# Autodesk Inventor assembly: Aufbau1,0
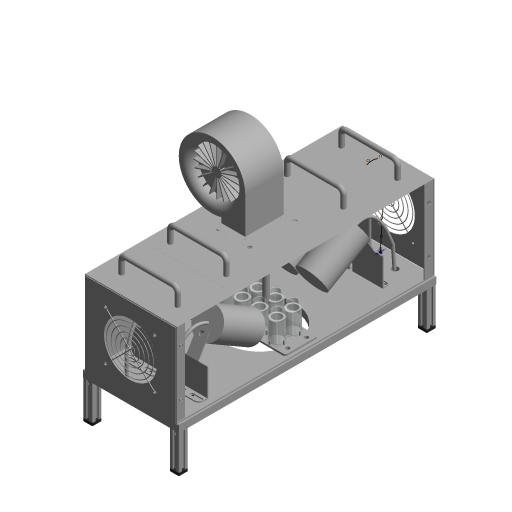
[picture p0: Inventor's stored thumbnail of the model, 512x512]
Saved by Autodesk Inventor 2024 (Build 280153000, 153)
## iProperties
Created: 2021-10-11
Part Number: Aufbau1,0
Document SubType Name: Baugruppe
Designer: bhelg
Author: bhelg
## Documents named in this file (20)
- E:\UV Reaktor 2\Aufbau 2,0.iam
- E:\UV Reaktor 2\Lampe.ipt
- E:\UV Reaktor 2\Glas klein.ipt
- E:\UV Reaktor 2\Grundplatte 2,0.ipt
- E:\UV Reaktor 2\Lampenhalterung 2,0.ipt
- E:\UV Reaktor 2\Halterung Gläser D27.4.ipt
- E:\UV Reaktor 2\Wobatech Abdeckkappe 20x20.ipt
- E:\UV Reaktor 2\20x20Profil 1.0.ipt
- E:\UV Reaktor 2\Deckel1,0.ipt
- E:\UV Reaktor 2\Seitenplatte 1,0.ipt
- E:\UV Reaktor 2\Sensormechanismus\Stativstange.ipt
- E:\UV Reaktor 2\Sensormechanismus\Stellring.ipt
- E:\UV Reaktor 2\Sensormechanismus\Arm.ipt
- E:\UV Reaktor 2\Sensormechanismus\Glashalter.ipt
- E:\UV Reaktor 2\Sensormechanismus\Glas.ipt
- E:\UV Reaktor 2\Blechgriff.ipt
- E:\UV Reaktor 2\Deckelanschlag.ipt
- E:\UV Reaktor 2\Deckel 2,0.ipt
- E:\UV Reaktor 2\Lüfter G1G108-AB17-02 1,0.ipt
- E:\UV Reaktor 2\Lüftergitter 1,0.ipt
## Components (45 placed, 19 different names)
1. Grundplatte 2,0:1 — Fluchtend:1, Fluchtend:2, Fluchtend:3, Passend:1, Winkel:1, Passend:3, Winkel:2, Einfügen:3, Tangential:1, Passend:8, Passend:9, Passend:10, Winkel:3, Winkel:4, Winkel:5, Tangential:2, Tangential:3, Tangential:4, Passend:22, Passend:23, Passend:24, Passend:25, Einfügen:19, Einfügen:20, Einfügen:21, Einfügen:22, Winkel:6, Passend:31, Passend:32, Winkel:7, Winkel:8, Einfügen:25, Fluchtend:5, Fluchtend:6
2. Lampenhalterung 2,0:1 — Passend:1, Passend:2, Winkel:1, Einfügen:2, Passend:5, Passend:6, Passend:7, Tangential:1
3. Lampe:1 — Passend:2, Einfügen:2, Passend:5, Passend:6, Passend:7
4. Halterung Gläser D27.4:1 — Passend:3, Winkel:2, Einfügen:3, Passend:4, Passend:15, Passend:16, Passend:17, Passend:18, Passend:19, Passend:20, Passend:21, Einfügen:7, Einfügen:8, Einfügen:9, Einfügen:10, Einfügen:11, Einfügen:12, Einfügen:13, Einfügen:14, Passend:47, Einfügen:28
5. Glas klein:1 — Passend:4, Einfügen:8
6. Lampe:2 — Passend:14, Einfügen:4
7. Lampe:3 — Passend:12, Einfügen:6
8. Lampe:4 — Passend:13, Einfügen:5
9. Lampenhalterung 2,0:2 — Passend:10, Winkel:5, Tangential:3, Passend:13, Einfügen:5
10. Lampenhalterung 2,0:3 — Passend:9, Winkel:3, Tangential:2, Passend:14, Einfügen:4
11. Lampenhalterung 2,0:4 — Passend:8, Winkel:4, Tangential:4, Passend:12, Einfügen:6
12. Glas klein:2 — Passend:17, Einfügen:14
13. Glas klein:3 — Passend:19, Einfügen:10
14. Glas klein:4 — Passend:18, Einfügen:13
15. Glas klein:5 — Passend:16, Einfügen:12
16. Glas klein:6 — Passend:20, Einfügen:9
17. Glas klein:7 — Passend:15, Einfügen:11
18. Glas klein:8 — Passend:21, Einfügen:7
19. Glas klein:9 — Passend:47, Einfügen:28
20. Wobatech Abdeckkappe 20x20:1 — Passend:26, Einfügen:15
21. Wobatech Abdeckkappe 20x20:2 — Passend:29, Einfügen:17
22. Wobatech Abdeckkappe 20x20:3 — Passend:28, Einfügen:16
23. Wobatech Abdeckkappe 20x20:4 — Passend:27, Einfügen:18
24. 20x20Profil 1.0:1 — Passend:22, Passend:26, Einfügen:15, Einfügen:21
25. 20x20Profil 1.0:2 — Passend:23, Passend:27, Einfügen:18, Einfügen:19
26. 20x20Profil 1.0:3 — Passend:24, Einfügen:16, Einfügen:22
27. 20x20Profil 1.0:4 — Passend:25, Passend:28, Passend:29, Einfügen:17, Einfügen:20
28. Deckel1,0:1 — Winkel:6, Passend:31, Passend:32, Passend:33, Passend:34, Passend:41, Passend:42, Passend:43, Passend:44, Winkel:11, Passend:50, Passend:51, Winkel:13, Winkel:14, Einfügen:31, Einfügen:32, Einfügen:33, Einfügen:34, Passend:55, Passend:56, Mate:60
29. Seitenplatte 1,0:1 — Passend:33, Winkel:8, Passend:42, Passend:43, Einfügen:39, Einfügen:40
30. Seitenplatte 1,0:2 — Passend:34, Winkel:7, Passend:41, Passend:44, Einfügen:37, Einfügen:38
31. Stativstange:1 — Einfügen:25, Passend:45, Passend:46
32. Stellring:1 — Passend:45
33. Arm:1 — Passend:46, Einfügen:26
34. Glashalter:1 — Einfügen:26, Einfügen:27
35. Glas:1 — Einfügen:27
36. Blechgriff:1 — Winkel:11, Einfügen:30
37. Blechgriff:2 — Einfügen:29, Winkel:14
38. Blechgriff:3 — Passend:51, Einfügen:31, Einfügen:34
39. Blechgriff:4 — Passend:50, Einfügen:32, Einfügen:33
40. Deckel 2,0:1 — Winkel:13, Einfügen:29, Einfügen:30, Passend:53, Fluchtend:9, Fluchtend:11, Passend:54, Winkel:15, Fluchtend:12, Fluchtend:13, Passend:57, Passend:58, Passend:59, Mate:60, Mate:61, Mate:62
41. Deckelanschlag:2 — Passend:53, Fluchtend:9, Fluchtend:11
42. Deckelanschlag:3 — Passend:54, Winkel:15, Fluchtend:12, Fluchtend:13, Passend:55, Passend:56
43. Lüfter G1G108-AB17-02 1,0:1 — Passend:57, Passend:58, Passend:59, Mate:61, Mate:62
44. Lüftergitter 1,0:1 — Einfügen:37, Einfügen:38
45. Lüftergitter 1,0:2 — Einfügen:39, Einfügen:40
## Relationships (111: Mate 51, Insert 35, Angle 12, Flush 9, Tangent 4)
- Fluchtend:1 [Flush]: Grundplatte 2,0:1
- Fluchtend:2 [Flush]: Grundplatte 2,0:1
- Fluchtend:3 [Flush]: Grundplatte 2,0:1
- Passend:1 [Mate]: Grundplatte 2,0:1 ↔ Lampenhalterung 2,0:1
- Passend:2 [Mate]: Lampenhalterung 2,0:1 ↔ Lampe:1
- Winkel:1 [Angle] (0 deg): Grundplatte 2,0:1 ↔ Lampenhalterung 2,0:1
- Einfügen:2 [Insert]: Lampenhalterung 2,0:1 ↔ Lampe:1
- Passend:3 [Mate]: Grundplatte 2,0:1 ↔ Halterung Gläser D27.4:1
- Winkel:2 [Angle] (0 deg): Grundplatte 2,0:1 ↔ Halterung Gläser D27.4:1
- Einfügen:3 [Insert]: Grundplatte 2,0:1 ↔ Halterung Gläser D27.4:1
- Passend:4 [Mate]: Halterung Gläser D27.4:1 ↔ Glas klein:1
- Passend:5 [Mate]: Lampenhalterung 2,0:1 ↔ Lampe:1
- Passend:6 [Mate]: Lampenhalterung 2,0:1 ↔ Lampe:1
- Passend:7 [Mate]: Lampenhalterung 2,0:1 ↔ Lampe:1
- Tangential:1 (0.533 mm): Grundplatte 2,0:1 ↔ Lampenhalterung 2,0:1
- Passend:8 [Mate]: Grundplatte 2,0:1 ↔ Lampenhalterung 2,0:4
- Passend:9 [Mate]: Grundplatte 2,0:1 ↔ Lampenhalterung 2,0:3
- Passend:10 [Mate]: Grundplatte 2,0:1 ↔ Lampenhalterung 2,0:2
- Winkel:3 [Angle] (0 deg): Grundplatte 2,0:1 ↔ Lampenhalterung 2,0:3
- Winkel:4 [Angle] (180 deg): Grundplatte 2,0:1 ↔ Lampenhalterung 2,0:4
- Winkel:5 [Angle] (180 deg): Grundplatte 2,0:1 ↔ Lampenhalterung 2,0:2
- Tangential:2 (0.533 mm): Grundplatte 2,0:1 ↔ Lampenhalterung 2,0:3
- Tangential:3 (0.533 mm): Grundplatte 2,0:1 ↔ Lampenhalterung 2,0:2
- Tangential:4 (0.533 mm): Grundplatte 2,0:1 ↔ Lampenhalterung 2,0:4
- Passend:12 [Mate]: Lampe:3 ↔ Lampenhalterung 2,0:4
- Passend:13 [Mate]: Lampe:4 ↔ Lampenhalterung 2,0:2
- Passend:14 [Mate]: Lampe:2 ↔ Lampenhalterung 2,0:3
- Einfügen:4 [Insert]: Lampe:2 ↔ Lampenhalterung 2,0:3
- Einfügen:5 [Insert]: Lampe:4 ↔ Lampenhalterung 2,0:2
- Einfügen:6 [Insert]: Lampe:3 ↔ Lampenhalterung 2,0:4
- Passend:15 [Mate]: Halterung Gläser D27.4:1 ↔ Glas klein:7
- Passend:16 [Mate]: Halterung Gläser D27.4:1 ↔ Glas klein:5
- Passend:17 [Mate]: Halterung Gläser D27.4:1 ↔ Glas klein:2
- Passend:18 [Mate]: Halterung Gläser D27.4:1 ↔ Glas klein:4
- Passend:19 [Mate]: Halterung Gläser D27.4:1 ↔ Glas klein:3
- Passend:20 [Mate]: Halterung Gläser D27.4:1 ↔ Glas klein:6
- Passend:21 [Mate]: Halterung Gläser D27.4:1 ↔ Glas klein:8
- Einfügen:7 [Insert]: Halterung Gläser D27.4:1 ↔ Glas klein:8
- Einfügen:8 [Insert]: Halterung Gläser D27.4:1 ↔ Glas klein:1
- Einfügen:9 [Insert]: Halterung Gläser D27.4:1 ↔ Glas klein:6
- Einfügen:10 [Insert]: Halterung Gläser D27.4:1 ↔ Glas klein:3
- Einfügen:11 [Insert]: Halterung Gläser D27.4:1 ↔ Glas klein:7
- Einfügen:12 [Insert]: Halterung Gläser D27.4:1 ↔ Glas klein:5
- Einfügen:13 [Insert]: Halterung Gläser D27.4:1 ↔ Glas klein:4
- Einfügen:14 [Insert]: Halterung Gläser D27.4:1 ↔ Glas klein:2
- Passend:22 [Mate]: Grundplatte 2,0:1 ↔ 20x20Profil 1.0:1
- Passend:23 [Mate]: Grundplatte 2,0:1 ↔ 20x20Profil 1.0:2
- Passend:24 [Mate]: Grundplatte 2,0:1 ↔ 20x20Profil 1.0:3
- Passend:25 [Mate]: Grundplatte 2,0:1 ↔ 20x20Profil 1.0:4
- Passend:26 [Mate]: Wobatech Abdeckkappe 20x20:1 ↔ 20x20Profil 1.0:1
- Passend:27 [Mate]: Wobatech Abdeckkappe 20x20:4 ↔ 20x20Profil 1.0:2
- Passend:28 [Mate]: Wobatech Abdeckkappe 20x20:3 ↔ 20x20Profil 1.0:4
- Passend:29 [Mate]: Wobatech Abdeckkappe 20x20:2 ↔ 20x20Profil 1.0:4
- Einfügen:15 [Insert]: Wobatech Abdeckkappe 20x20:1 ↔ 20x20Profil 1.0:1
- Einfügen:16 [Insert]: Wobatech Abdeckkappe 20x20:3 ↔ 20x20Profil 1.0:3
- Einfügen:17 [Insert]: Wobatech Abdeckkappe 20x20:2 ↔ 20x20Profil 1.0:4
- Einfügen:18 [Insert]: Wobatech Abdeckkappe 20x20:4 ↔ 20x20Profil 1.0:2
- Einfügen:19 [Insert]: Grundplatte 2,0:1 ↔ 20x20Profil 1.0:2
- Einfügen:20 [Insert]: Grundplatte 2,0:1 ↔ 20x20Profil 1.0:4
- Einfügen:21 [Insert]: Grundplatte 2,0:1 ↔ 20x20Profil 1.0:1
- Einfügen:22 [Insert]: Grundplatte 2,0:1 ↔ 20x20Profil 1.0:3
- Winkel:6 [Angle] (0 deg): Grundplatte 2,0:1 ↔ Deckel1,0:1
- Passend:31 [Mate] (0.5 mm): Grundplatte 2,0:1 ↔ Deckel1,0:1
- Passend:32 [Mate]: Grundplatte 2,0:1 ↔ Deckel1,0:1
- Passend:33 [Mate]: Deckel1,0:1 ↔ Seitenplatte 1,0:1
- Passend:34 [Mate]: Deckel1,0:1 ↔ Seitenplatte 1,0:2
- Winkel:7 [Angle] (0 deg): Grundplatte 2,0:1 ↔ Seitenplatte 1,0:2
- Winkel:8 [Angle] (0 deg): Grundplatte 2,0:1 ↔ Seitenplatte 1,0:1
- Passend:41 [Mate]: Deckel1,0:1 ↔ Seitenplatte 1,0:2
- Passend:42 [Mate]: Deckel1,0:1 ↔ Seitenplatte 1,0:1
- Passend:43 [Mate]: Deckel1,0:1 ↔ Seitenplatte 1,0:1
- Passend:44 [Mate]: Deckel1,0:1 ↔ Seitenplatte 1,0:2
- Einfügen:25 [Insert] (-6 mm): Grundplatte 2,0:1 ↔ Stativstange:1
- Passend:45 [Mate]: Stativstange:1 ↔ Stellring:1
- Passend:46 [Mate]: Stativstange:1 ↔ Arm:1
- Einfügen:26 [Insert] (-9 mm): Arm:1 ↔ Glashalter:1
- Einfügen:27 [Insert]: Glashalter:1 ↔ Glas:1
- Fluchtend:5 [Flush] (2.649 mm): Grundplatte 2,0:1
- Fluchtend:6 [Flush] (-102.5 mm): Grundplatte 2,0:1
- Passend:47 [Mate]: Halterung Gläser D27.4:1 ↔ Glas klein:9
- Einfügen:28 [Insert]: Halterung Gläser D27.4:1 ↔ Glas klein:9
- Winkel:11 [Angle] (0 deg): Deckel1,0:1 ↔ Blechgriff:1
- Passend:50 [Mate]: Deckel1,0:1 ↔ Blechgriff:4
- Passend:51 [Mate]: Deckel1,0:1 ↔ Blechgriff:3
- Winkel:13 [Angle] (0 deg): Deckel1,0:1 ↔ Deckel 2,0:1
- Einfügen:29 [Insert]: Blechgriff:2 ↔ Deckel 2,0:1
- Einfügen:30 [Insert]: Blechgriff:1 ↔ Deckel 2,0:1
- Winkel:14 [Angle] (0 deg): Deckel1,0:1 ↔ Blechgriff:2
- Einfügen:31 [Insert]: Deckel1,0:1 ↔ Blechgriff:3
- Einfügen:32 [Insert]: Deckel1,0:1 ↔ Blechgriff:4
- Passend:53 [Mate]: Deckel 2,0:1 ↔ Deckelanschlag:2
- Fluchtend:9 [Flush] (4 mm): Deckel 2,0:1 ↔ Deckelanschlag:2
- Fluchtend:11 [Flush] (-7 mm): Deckel 2,0:1 ↔ Deckelanschlag:2
- Passend:54 [Mate]: Deckel 2,0:1 ↔ Deckelanschlag:3
- Winkel:15 [Angle] (180 deg): Deckel 2,0:1 ↔ Deckelanschlag:3
- Fluchtend:12 [Flush] (4 mm): Deckel 2,0:1 ↔ Deckelanschlag:3
- Fluchtend:13 [Flush] (-7 mm): Deckel 2,0:1 ↔ Deckelanschlag:3
- Einfügen:33 [Insert]: Deckel1,0:1 ↔ Blechgriff:4
- Einfügen:34 [Insert]: Deckel1,0:1 ↔ Blechgriff:3
- Passend:55 [Mate]: Deckel1,0:1 ↔ Deckelanschlag:3
- Passend:56 [Mate]: Deckel1,0:1 ↔ Deckelanschlag:3
- Einfügen:37 [Insert]: Seitenplatte 1,0:2 ↔ Lüftergitter 1,0:1
- Einfügen:38 [Insert]: Seitenplatte 1,0:2 ↔ Lüftergitter 1,0:1
- Einfügen:39 [Insert]: Seitenplatte 1,0:1 ↔ Lüftergitter 1,0:2
- Einfügen:40 [Insert]: Seitenplatte 1,0:1 ↔ Lüftergitter 1,0:2
- Passend:57 [Mate]: Deckel 2,0:1 ↔ Lüfter G1G108-AB17-02 1,0:1
- Passend:58 [Mate]: Deckel 2,0:1 ↔ Lüfter G1G108-AB17-02 1,0:1
- Passend:59 [Mate] (30 mm): Deckel 2,0:1 ↔ Lüfter G1G108-AB17-02 1,0:1
- Mate:60: Deckel1,0:1 ↔ Deckel 2,0:1
- Mate:61: Deckel 2,0:1 ↔ Lüfter G1G108-AB17-02 1,0:1
- Mate:62: Deckel 2,0:1 ↔ Lüfter G1G108-AB17-02 1,0:1
